# Autodesk Inventor assembly: Fixture Assembly
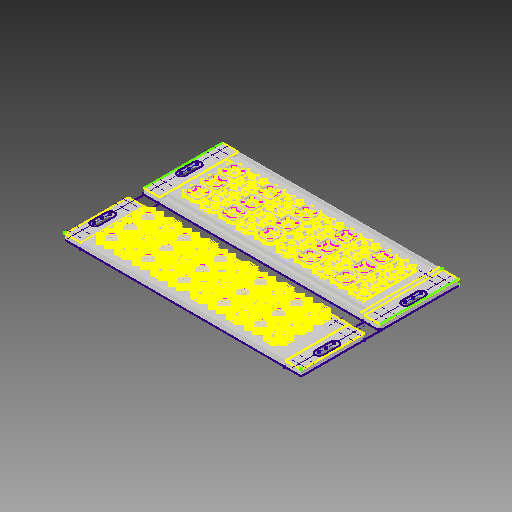
[picture p0: Inventor's stored thumbnail of the model, 512x512]
Saved by Autodesk Inventor 2018 (Build 220112000, 112)
## iProperties
Created: 2016-04-08
Part Number: Fixture Assembly
Document SubType Name: Assembly
Designer: Sam Clay
Author: Sam Clay
## Documents named in this file (6)
- Z:\enclosure\inventor\Fixture Assembly.iam
- Z:\enclosure\inventor\Fixture Base.ipt
- Z:\enclosure\inventor\Case Top Contour Fixture.ipt
- Z:\enclosure\inventor\Case Bottom Contour Fixture.ipt
- Z:\enclosure\inventor\Case Top Pocket Fixture.ipt
- Z:\enclosure\inventor\Case Bottom Pocket Fixture.ipt
## Components (61 placed, 5 different names)
1. Fixture Base:1 — Mate:26, Mate:27, Mate:28, Mate:35, Mate:36, Mate:38, Mate:43
2. Case Top Contour Fixture:1 — Mate:26, Mate:27, Mate:28, Mate:31, Mate:32, Mate:29
3. Case Top Contour Fixture:2
4. Case Top Contour Fixture:3
5. Case Top Contour Fixture:4
6. Case Top Contour Fixture:5
7. Case Top Contour Fixture:6
8. Case Top Contour Fixture:7 — Mate:23
9. Case Top Contour Fixture:8
10. Case Top Contour Fixture:9
11. Case Bottom Contour Fixture:7 — Mate:21, Mate:22, Mate:23, Mate:29
12. Case Bottom Contour Fixture:8
13. Case Bottom Contour Fixture:9
14. Case Bottom Contour Fixture:10
15. Case Bottom Contour Fixture:11
16. Case Bottom Contour Fixture:12
17. Case Bottom Contour Fixture:13
18. Case Bottom Contour Fixture:14
19. Case Bottom Contour Fixture:15
20. Case Top Contour Fixture:10 — Mate:21, Mate:22
21. Case Top Contour Fixture:11
22. Case Top Contour Fixture:12
23. Case Top Contour Fixture:13
24. Case Top Contour Fixture:14
25. Case Top Contour Fixture:15
26. Case Bottom Contour Fixture:16 — Mate:31, Mate:32
27. Case Bottom Contour Fixture:17
28. Case Bottom Contour Fixture:18
29. Case Bottom Contour Fixture:19
30. Case Bottom Contour Fixture:20
31. Case Bottom Contour Fixture:21
32. Case Top Pocket Fixture:1 — Mate:34, Mate:35, Mate:36, Mate:39, Mate:41, Mate:42
33. Case Top Pocket Fixture:3
34. Case Top Pocket Fixture:4
35. Case Top Pocket Fixture:5
36. Case Top Pocket Fixture:6
37. Case Top Pocket Fixture:7
38. Case Top Pocket Fixture:8
39. Case Top Pocket Fixture:9
40. Case Top Pocket Fixture:10
41. Case Bottom Pocket Fixture:1 — Mate:34, Mate:38, Mate:39
42. Case Bottom Pocket Fixture:3
43. Case Bottom Pocket Fixture:4
44. Case Bottom Pocket Fixture:5
45. Case Bottom Pocket Fixture:6
46. Case Bottom Pocket Fixture:7
47. Case Bottom Pocket Fixture:2 — Mate:40, Mate:43, Mate:41, Mate:44
48. Case Bottom Pocket Fixture:8
49. Case Bottom Pocket Fixture:9
50. Case Bottom Pocket Fixture:10
51. Case Bottom Pocket Fixture:11
52. Case Bottom Pocket Fixture:12
53. Case Bottom Pocket Fixture:13
54. Case Bottom Pocket Fixture:14
55. Case Bottom Pocket Fixture:15
56. Case Top Pocket Fixture:2 — Mate:40, Mate:42, Mate:44
57. Case Top Pocket Fixture:11
58. Case Top Pocket Fixture:12
59. Case Top Pocket Fixture:13
60. Case Top Pocket Fixture:14
61. Case Top Pocket Fixture:15
## Component patterns: (9 elements, first: Case Top Contour Fixture:1), (9 elements, first: Case Bottom Contour Fixture:7), (6 elements, first: Case Top Contour Fixture:10), (6 elements, first: Case Bottom Contour Fixture:16), (9 elements, first: Case Top Pocket Fixture:1), (6 elements, first: Case Bottom Pocket Fixture:1), (9 elements, first: Case Bottom Pocket Fixture:2), (6 elements, first: Case Top Pocket Fixture:2)
## Relationships (19: Mate 19)
- Mate:21: Case Bottom Contour Fixture:7 ↔ Case Top Contour Fixture:10
- Mate:22 (6.604 mm): Case Bottom Contour Fixture:7 ↔ Case Top Contour Fixture:10
- Mate:23: Case Top Contour Fixture:7 ↔ Case Bottom Contour Fixture:7
- Mate:26 (16.51 mm): Fixture Base:1 ↔ Case Top Contour Fixture:1
- Mate:27 (24.13 mm): Fixture Base:1 ↔ Case Top Contour Fixture:1
- Mate:28 (41.91 mm): Fixture Base:1 ↔ Case Top Contour Fixture:1
- Mate:29 (304.8 mm): Case Top Contour Fixture:1 ↔ Case Bottom Contour Fixture:7
- Mate:31: Case Top Contour Fixture:1 ↔ Case Bottom Contour Fixture:16
- Mate:32 (6.604 mm): Case Top Contour Fixture:1 ↔ Case Bottom Contour Fixture:16
- Mate:34: Case Top Pocket Fixture:1 ↔ Case Bottom Pocket Fixture:1
- Mate:35 (3.175 mm): Fixture Base:1 ↔ Case Top Pocket Fixture:1
- Mate:36 (1.27 mm): Fixture Base:1 ↔ Case Top Pocket Fixture:1
- Mate:38: Fixture Base:1 ↔ Case Bottom Pocket Fixture:1
- Mate:39 (6.604 mm): Case Top Pocket Fixture:1 ↔ Case Bottom Pocket Fixture:1
- Mate:40: Case Bottom Pocket Fixture:2 ↔ Case Top Pocket Fixture:2
- Mate:41 (304.8 mm): Case Top Pocket Fixture:1 ↔ Case Bottom Pocket Fixture:2
- Mate:42: Case Top Pocket Fixture:1 ↔ Case Top Pocket Fixture:2
- Mate:43: Fixture Base:1 ↔ Case Bottom Pocket Fixture:2
- Mate:44 (6.604 mm): Case Bottom Pocket Fixture:2 ↔ Case Top Pocket Fixture:2
